# Autodesk Inventor assembly: 1.7assem
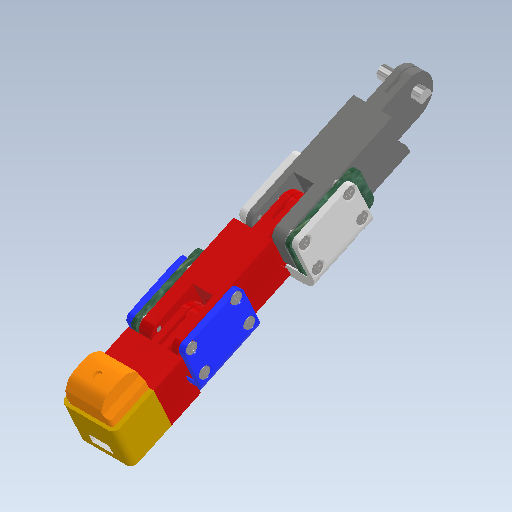
[picture p0: Inventor's stored thumbnail of the model, 512x512]
Saved by Autodesk Inventor 2020 (Build 240168000, 168)
## iProperties
Created: 2020-01-20
Part Number: 1.7assem
Document SubType Name: Assembly
Designer: sami_
Author: sami_
## Documents named in this file (4)
- C:\Users\sami_\Documents\V1.6\Workgroups\NotInProject\RING\finger RING.iam
- C:\Users\sami_\Documents\V1.6\RingL1.iam
- C:\Users\sami_\Documents\V1.6\RingL2.iam
- C:\Users\sami_\Documents\V1.6\RingL3.iam
## Components (3 placed, 3 different names)
1. RingL1:1 [sub-assembly]
2. RingL2:1 [sub-assembly]
3. RingL3:1 [sub-assembly]
## Relationships (3: RevoluteJoint 2, Mate 1)
- [RevoluteJoint]: RingL1:1 ↔ RingL2:1
- [Mate]: RingL1:1 ↔ RingL2:1
- [RevoluteJoint]: RingL2:1 ↔ RingL3:1
